# Autodesk Inventor assembly: lw_6_сборка
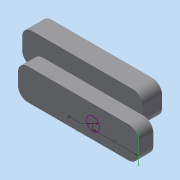
[picture p0: Inventor's stored thumbnail of the model, 180x180]
Saved by Autodesk Inventor 2019 (Build 230136000, 136)
## iProperties
Created: 2021-05-14
Part Number: lw_6_сборка
Material: Типовые
Document SubType Name: Assembly
Designer: Kurbatova
Author: Kurbatova
## Documents named in this file (3)
- C:\Users\Kurbatova\source\LW2021\LW_SAPR\Сборки\lw_6_сборка.iam
- C:\Users\Kurbatova\source\LW2021\LW_SAPR\Детали\lw_6_part1.ipt
- C:\Users\Kurbatova\source\LW2021\LW_SAPR\Детали\lw_6_part2.ipt
## Components (2 placed, 2 different names)
1. lw_6_part1:1 — Совмещение:1
2. lw_6_part2:1 — Совмещение:1
## Relationships (1: Mate 1)
- Совмещение:1 [Mate]: lw_6_part1:1 ↔ lw_6_part2:1
